# Autodesk Inventor assembly: Case Top
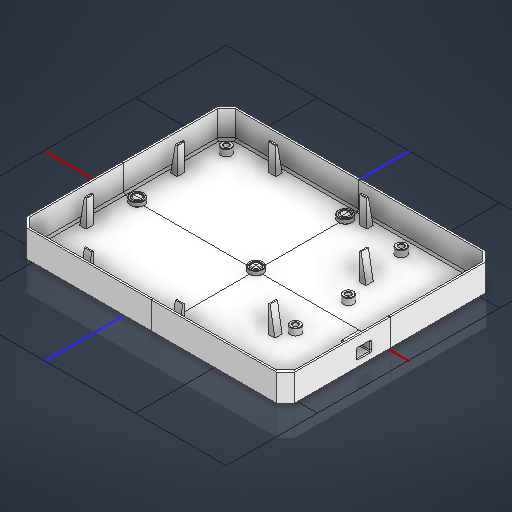
[picture p0: Inventor's stored thumbnail of the model, 512x512]
Saved by Autodesk Inventor 2026 (Build 300175000, 175)
## iProperties
Created: 2025-06-07
Part Number: Case Top
Document SubType Name: Assembly
Designer: ckyiu
Author: ckyiu
## Documents named in this file (3)
- F:\Chessboard-Design\Assemblies\Case\Case Top.iam
- F:\Chessboard-Design\Parts\Case\Case Bottom.ipt
- F:\Chessboard-Design\Parts\Case\Case Bottom Ring.ipt
## Components (6 placed, 2 different names)
1. Case Bottom:1 — Insert:1, Insert:2, Insert:3, Insert:4, Insert:5
2. Case Bottom Ring:1 — Insert:1
3. Case Bottom Ring:2 — Insert:2
4. Case Bottom Ring:3 — Insert:3
5. Case Bottom Ring:4 — Insert:4
6. Case Bottom Ring:5 — Insert:5
## Relationships (5: Insert 5)
- Insert:1: Case Bottom:1 ↔ Case Bottom Ring:1
- Insert:2: Case Bottom:1 ↔ Case Bottom Ring:2
- Insert:3: Case Bottom:1 ↔ Case Bottom Ring:3
- Insert:4: Case Bottom:1 ↔ Case Bottom Ring:4
- Insert:5: Case Bottom:1 ↔ Case Bottom Ring:5
